# Autodesk Inventor assembly: caja sensora
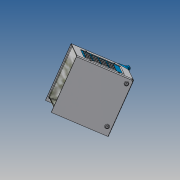
[picture p0: Inventor's stored thumbnail of the model, 180x180]
Saved by Autodesk Inventor 2017 (Build 210142000, 142)
## iProperties
Part Number: caja sensora
Material: Genérico
Document SubType Name: Assembly
Designer: Leo
Author: Leo
## Documents named in this file (6)
- C:\Users\Leo\Dropbox\multiactuador\caja sensora.iam
- C:\Users\Leo\Dropbox\multiactuador\case.iam
- C:\Users\Leo\Dropbox\multiactuador\placa.iam
- C:\Users\Leo\Dropbox\multiactuador\componentes\botonera.ipt
- C:\Users\Leo\Dropbox\multiactuador\componentes\mb1010.ipt
- C:\Users\Leo\Dropbox\multiactuador\caja sensora\Design Accelerator\Bolted Connection1.iam
## Components (5 placed, 5 different names)
1. case:1 [sub-assembly] — Coincidencia:3, Coincidencia:2, Coincidencia:4, Coincidencia:5, Coincidencia:6, Coincidencia:7, Insert:11
2. placa:1 [sub-assembly] — Coincidencia:3, Coincidencia:2, Coincidencia:4, Mate:8, Mate:9
3. botonera:1 — Coincidencia:5, Coincidencia:6, Coincidencia:7
4. mb1010:1 — Insert:11
5. Bolted Connection:1 [sub-assembly] — Mate:8, Mate:9
## Relationships (9: Mate 8, Insert 1)
- Coincidencia:3 [Mate]: case:1 ↔ placa:1
- Coincidencia:2 [Mate] (10 mm): case:1 ↔ placa:1
- Coincidencia:4 [Mate] (2 mm): case:1 ↔ placa:1
- Coincidencia:5 [Mate]: case:1 ↔ botonera:1
- Coincidencia:6 [Mate] (-2.5 mm): case:1 ↔ botonera:1
- Coincidencia:7 [Mate]: case:1 ↔ botonera:1
- Mate:8: placa:1 ↔ Bolted Connection:1
- Mate:9: placa:1 ↔ Bolted Connection:1
- Insert:11 (6 mm): case:1 ↔ mb1010:1
